# Autodesk Inventor assembly: wiper_assembly
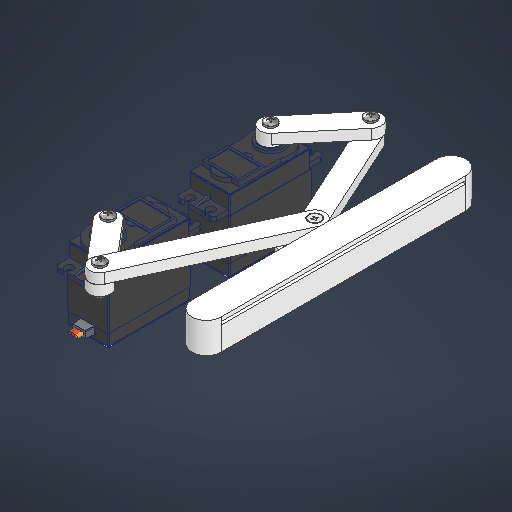
[picture p0: Inventor's stored thumbnail of the model, 512x512]
Saved by Autodesk Inventor 2026.2 (Build 302298000, 298)
## iProperties
Created: 2026-03-27
Part Number: wiper_assembly
Document SubType Name: Assembly
Designer: Tathagata Sikdar
Author: Tathagata Sikdar
## Documents named in this file (8)
- D:\Productivity\Repos\early-lameness-detection\inventor_models\wiper_assembly.iam
- D:\Productivity\Repos\early-lameness-detection\inventor_models\wiper_linkage_middle_arm.ipt
- D:\Productivity\Repos\early-lameness-detection\inventor_models\wiper_linkage_motor_connect.ipt
- D:\Productivity\Repos\early-lameness-detection\inventor_models\wiper_linkage_magnet_holder.ipt
- D:\Productivity\Repos\early-lameness-detection\inventor_models\mcmaster_carr\91828A211_Corrosion-Resistant 18-8 Stainless Steel Hex Nut\91828A211_Corrosion-Resistant 18-8 Stainless Steel Hex Nut\91828A211_Corro.ipt
- D:\Productivity\Repos\early-lameness-detection\inventor_models\mcmaster_carr\92000A124_Passivated 18-8 Stainless Steel Pan Head Phillips Screws\92000A124_Passivated 18-8 Stainless Steel Pan Head Phillips Screws.ipt
- D:\Productivity\Repos\early-lameness-detection\inventor_models\mg996r-servo-motor-1.snapshot.7\MG996R SERVO\MG996R SBORKA\MG996R SBORKA\MG996R SBORKA.ipt
- D:\Productivity\Repos\early-lameness-detection\inventor_models\mcmaster_carr\92010A120_Passivated 18-8 Stainless Steel Phillips Flat Head Screw\92010A120_Passivated 18-8 Stainless Steel Phillips Flat Head Screw.ipt
## Components (17 placed, 7 different names)
1. wiper_linkage_motor_connect:1 — Mate:10, Mate:11, Mate:15, Mate:16, Mate:17, Insert:6, Insert:9, Insert:16
2. wiper_linkage_motor_connect:2 — Mate:14, Mate:16, Insert:4, Insert:7, Insert:18, Insert:28
3. wiper_linkage_magnet_holder:1 — Angle:1, Insert:12, Insert:17, Insert:26, Insert:27
4. wiper_linkage_middle_arm:1 — Mate:10, Mate:11, Insert:5, Insert:12, Insert:24
5. wiper_linkage_middle_arm:2 — Insert:17, Insert:18, Insert:19, Insert:25
6. 92000A124_Passivated 18-8 Stainless Steel Pan Head Phillips Screws:1 — Insert:6
7. 92000A124_Passivated 18-8 Stainless Steel Pan Head Phillips Screws:2 — Insert:5
8. 92000A124_Passivated 18-8 Stainless Steel Pan Head Phillips Screws:3 — Insert:7
9. 92000A124_Passivated 18-8 Stainless Steel Pan Head Phillips Screws:6 — Insert:4
10. 91828A211_Corro:3 — Insert:9
11. 91828A211_Corro:4 — Insert:19
12. MG996R SBORKA:1 — Flush:1, Insert:16, Flush:2
13. MG996R SBORKA:2 — Flush:1, Insert:28
14. 92010A120_Passivated 18-8 Stainless Steel Phillips Flat Head Screw:1 — Insert:24
15. 92010A120_Passivated 18-8 Stainless Steel Phillips Flat Head Screw:2 — Insert:25
16. 91828A211_Corro:5 — Insert:26
17. 91828A211_Corro:6 — Insert:27
## Relationships (24: Insert 15, Mate 6, Flush 2, Angle 1)
- Mate:10: wiper_linkage_motor_connect:1 ↔ wiper_linkage_middle_arm:1
- Mate:11: wiper_linkage_motor_connect:1 ↔ wiper_linkage_middle_arm:1
- Mate:14: wiper_linkage_motor_connect:2
- Mate:15: wiper_linkage_motor_connect:1
- Mate:16 (-80 mm): wiper_linkage_motor_connect:1 ↔ wiper_linkage_motor_connect:2
- Mate:17: wiper_linkage_motor_connect:1
- Angle:1 (180 deg): wiper_linkage_magnet_holder:1
- Insert:4: wiper_linkage_motor_connect:2 ↔ 92000A124_Passivated 18-8 Stainless Steel Pan Head Phillips Screws:6
- Insert:5: wiper_linkage_middle_arm:1 ↔ 92000A124_Passivated 18-8 Stainless Steel Pan Head Phillips Screws:2
- Insert:6: wiper_linkage_motor_connect:1 ↔ 92000A124_Passivated 18-8 Stainless Steel Pan Head Phillips Screws:1
- Insert:7: wiper_linkage_motor_connect:2 ↔ 92000A124_Passivated 18-8 Stainless Steel Pan Head Phillips Screws:3
- Insert:9: wiper_linkage_motor_connect:1 ↔ 91828A211_Corro:3
- Insert:12: wiper_linkage_magnet_holder:1 ↔ wiper_linkage_middle_arm:1
- Flush:1: MG996R SBORKA:1 ↔ MG996R SBORKA:2
- Insert:16: wiper_linkage_motor_connect:1 ↔ MG996R SBORKA:1
- Flush:2: MG996R SBORKA:1
- Insert:17: wiper_linkage_magnet_holder:1 ↔ wiper_linkage_middle_arm:2
- Insert:18: wiper_linkage_motor_connect:2 ↔ wiper_linkage_middle_arm:2
- Insert:19: wiper_linkage_middle_arm:2 ↔ 91828A211_Corro:4
- Insert:24: wiper_linkage_middle_arm:1 ↔ 92010A120_Passivated 18-8 Stainless Steel Phillips Flat Head Screw:1
- Insert:25: wiper_linkage_middle_arm:2 ↔ 92010A120_Passivated 18-8 Stainless Steel Phillips Flat Head Screw:2
- Insert:26: wiper_linkage_magnet_holder:1 ↔ 91828A211_Corro:5
- Insert:27: wiper_linkage_magnet_holder:1 ↔ 91828A211_Corro:6
- Insert:28: wiper_linkage_motor_connect:2 ↔ MG996R SBORKA:2
